# Autodesk Inventor assembly: PMAsm
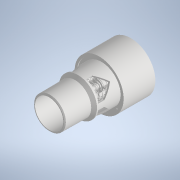
[picture p0: Inventor's stored thumbnail of the model, 180x180]
Saved by Autodesk Inventor 2020 (Build 240168000, 168)
## iProperties
Created: 2020-05-07
Part Number: PMAsm
Document SubType Name: Assembly
Designer: Theo Cominotto
Author: Theo Cominotto
## Documents named in this file (6)
- C:\Users\Theo Cominotto\Dropbox\Beademingstoestel VUB\Beademingstoestel VUB-PEEP VALVE\Peep Mimic\PMAsm.iam
- C:\Users\Theo Cominotto\Dropbox\Beademingstoestel VUB\Beademingstoestel VUB-PEEP VALVE\Peep Mimic\PMBase.ipt
- C:\Users\Theo Cominotto\Dropbox\Beademingstoestel VUB\Beademingstoestel VUB-PEEP VALVE\Peep Mimic\PMCover.ipt
- C:\Users\Theo Cominotto\Dropbox\Beademingstoestel VUB\Beademingstoestel VUB-PEEP VALVE\Peep Mimic\PMSeal.ipt
- C:\Users\Theo Cominotto\Dropbox\Beademingstoestel VUB\Beademingstoestel VUB-PEEP VALVE\Peep Mimic\TaperedSpring.ipt
- C:\Users\Theo Cominotto\Dropbox\Beademingstoestel VUB\Beademingstoestel VUB-PEEP VALVE\Peep Mimic\CylindricalSpring.ipt
## Components (5 placed, 5 different names)
1. PMBase:1 — Mate:1, Mate:2, Mate:4, Mate:5
2. PMCover:1 — Mate:2, Mate:3, Mate:5, Mate:6, Mate:7, Mate:8
3. PMSeal:1 — Mate:3, Mate:4, Mate:9
4. TaperedSpring:1 — Mate:8, Mate:9
5. CylindricalSpring:1 — Mate:6, Mate:7
## Relationships (9: Mate 9)
- Mate:1: PMBase:1
- Mate:2: PMBase:1 ↔ PMCover:1
- Mate:3: PMCover:1 ↔ PMSeal:1
- Mate:4: PMBase:1 ↔ PMSeal:1
- Mate:5 (13.697 mm): PMBase:1 ↔ PMCover:1
- Mate:6: PMCover:1 ↔ CylindricalSpring:1
- Mate:7: PMCover:1 ↔ CylindricalSpring:1
- Mate:8: PMCover:1 ↔ TaperedSpring:1
- Mate:9: PMSeal:1 ↔ TaperedSpring:1
